# Autodesk Inventor assembly: HbSocketU03
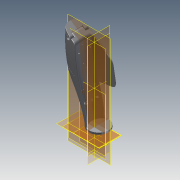
[picture p0: Inventor's stored thumbnail of the model, 180x180]
Saved by Autodesk Inventor 2015 SP1 (Build 190203100, 203)
## iProperties
Created: 2015-08-03
Part Number: HbSocketU03
Document SubType Name: Assembly
Designer: Yamaura
Author: Yamaura
## Documents named in this file (7)
- C:\Users\Yamaura\Documents\GitHub\HACKberry\HACKberry-hardware\3D\Inventor\Parts\HbSocketU03.iam
- C:\Users\Yamaura\Documents\GitHub\HACKberry\HACKberry-hardware\3D\Inventor\Parts\HbMainFrameB03.ipt
- C:\Users\Yamaura\Documents\GitHub\HACKberry\HACKberry-hardware\3D\Inventor\Parts\HbMainFrameA03.ipt
- C:\Users\Yamaura\Documents\GitHub\HACKberry\HACKberry-hardware\3D\Inventor\Parts\HbBatteryCase03.ipt
- C:\Users\Yamaura\Documents\GitHub\HACKberry\HACKberry-hardware\3D\Inventor\Parts\HbBatteryLockKnob01.ipt
- C:\Users\Yamaura\Documents\GitHub\HACKberry\HACKberry-hardware\3D\Inventor\Parts\HbBatteryDoorB03.ipt
- C:\Users\Yamaura\Documents\GitHub\HACKberry\HACKberry-hardware\3D\Inventor\Parts\HbBatteryDoorA03.ipt
## Components (6 placed, 6 different names)
1. HbMainFrameA03:1 — フラッシュ:1, フラッシュ:3, メイト:1, メイト:2, メイト:3, メイト:8
2. HbMainFrameB03:1 — メイト:2, メイト:3, メイト:4, メイト:5, メイト:6, メイト:7, メイト:8, 角度:1, メイト:10, メイト:11
3. HbBatteryCase03:1 — メイト:4, メイト:5, メイト:6, メイト:9
4. HbBatteryLockKnob01:1 — メイト:7, 角度:1, メイト:9
5. HbBatteryDoorB03:1 — メイト:10, メイト:11, メイト:12, メイト:13, メイト:14
6. HbBatteryDoorA03:1 — メイト:12, メイト:13, メイト:14, 角度:2
## Relationships (18: Mate 14, Flush 2, Angle 2)
- フラッシュ:1 [Flush]: HbMainFrameA03:1
- フラッシュ:3 [Flush]: HbMainFrameA03:1
- メイト:1 [Mate]: HbMainFrameA03:1
- メイト:2 [Mate]: HbMainFrameA03:1 ↔ HbMainFrameB03:1
- メイト:3 [Mate]: HbMainFrameA03:1 ↔ HbMainFrameB03:1
- メイト:4 [Mate]: HbMainFrameB03:1 ↔ HbBatteryCase03:1
- メイト:5 [Mate]: HbMainFrameB03:1 ↔ HbBatteryCase03:1
- メイト:6 [Mate]: HbMainFrameB03:1 ↔ HbBatteryCase03:1
- メイト:7 [Mate]: HbMainFrameB03:1 ↔ HbBatteryLockKnob01:1
- メイト:8 [Mate]: HbMainFrameA03:1 ↔ HbMainFrameB03:1
- 角度:1 [Angle] (180 deg): HbMainFrameB03:1 ↔ HbBatteryLockKnob01:1
- メイト:9 [Mate]: HbBatteryCase03:1 ↔ HbBatteryLockKnob01:1
- メイト:10 [Mate]: HbMainFrameB03:1 ↔ HbBatteryDoorB03:1
- メイト:11 [Mate] (0.3 mm): HbMainFrameB03:1 ↔ HbBatteryDoorB03:1
- メイト:12 [Mate]: HbBatteryDoorB03:1 ↔ HbBatteryDoorA03:1
- メイト:13 [Mate]: HbBatteryDoorB03:1 ↔ HbBatteryDoorA03:1
- メイト:14 [Mate]: HbBatteryDoorB03:1 ↔ HbBatteryDoorA03:1
- 角度:2 [Angle] (0 deg): HbBatteryDoorA03:1
